# Autodesk Inventor assembly: Manipulator
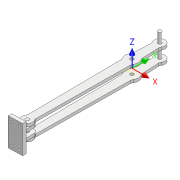
[picture p0: Inventor's stored thumbnail of the model, 180x180]
Saved by Autodesk Inventor 2020 (Build 240168000, 168)
## iProperties
Created: 2020-03-27
Part Number: Manipulator
Document SubType Name: Assembly
Designer: JakubTomaszewski
Mass: 37.9991 g
Surface Area: 185.846 cm^2
Volume: 27.2551 cm^3
Density: 1.3942 g/cm^3
Author: JakubTomaszewski
## Documents named in this file (5)
- C:\Users\JakubTomaszewski\Documents\Inventor\Manipulator\TrzecieOgniwo.iam
- C:\Users\JakubTomaszewski\Documents\Inventor\Manipulator\Ogniwo2_lacznik.ipt
- C:\Users\JakubTomaszewski\Documents\Inventor\Manipulator\Ogniwo2.ipt
- C:\Users\JakubTomaszewski\Documents\Inventor\Manipulator\Ogniwo2.2_lacznik.ipt
- C:\Users\JakubTomaszewski\Documents\Inventor\Manipulator\Efektor.ipt
## Components (5 placed, 4 different names)
1. Ogniwo2_lacznik:1 — Ogniwo2_2_2
2. Ogniwo2:1 — Lacznik2_2, Obrotowe:36, Równoległe:1, Równoległe:2, Równoległe:3
3. Ogniwo2:2 — Ogniwo2_2_2, Lacznik2_1
4. Ogniwo2.2_lacznik:1 — Lacznik2_1, Lacznik2_2
5. Efektor:1 — Obrotowe:36
## Relationships (7: WeldJoint 3, Flush 3, RevoluteJoint 1)
- Ogniwo2_2_2 [WeldJoint]: Ogniwo2_lacznik:1 ↔ Ogniwo2:2
- Lacznik2_1 [WeldJoint]: Ogniwo2:2 ↔ Ogniwo2.2_lacznik:1
- Lacznik2_2 [WeldJoint]: Ogniwo2:1 ↔ Ogniwo2.2_lacznik:1
- Obrotowe:36 [RevoluteJoint]: Ogniwo2:1 ↔ Efektor:1
- Równoległe:1 [Flush]: Ogniwo2:1
- Równoległe:2 [Flush]: Ogniwo2:1
- Równoległe:3 [Flush]: Ogniwo2:1
